# Autodesk Inventor assembly: Ensamblaje Alison Martínez 1190119
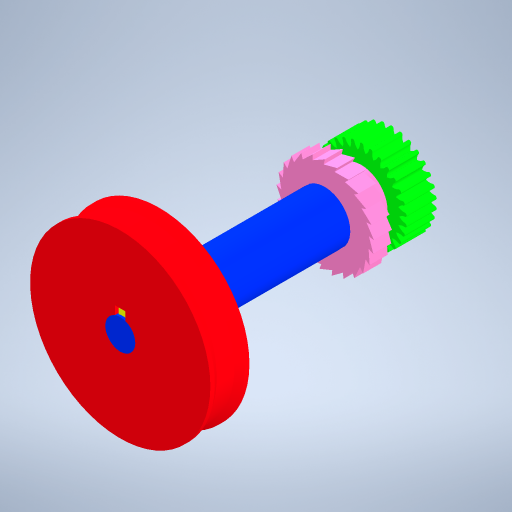
[picture p0: Inventor's stored thumbnail of the model, 512x512]
Saved by Autodesk Inventor 2024 (Build 280153000, 153)
## iProperties
Created: 2024-03-25
Part Number: Ensamblaje Alison Martínez 1190119
Document SubType Name: Assembly
Designer: Alison
Author: Alison
## Documents named in this file (6)
- C:\Users\Alison\Documents\Inventario\Ensamblaje Alison Martínez 1190119.iam
- C:\Users\Alison\Downloads\POLEA.ipt
- C:\Users\Alison\Downloads\ENGRANE.ipt
- C:\Users\Alison\Downloads\EJE_CUÑEROS.ipt
- C:\Users\Alison\Downloads\CUÑA.ipt
- C:\Users\Alison\Documents\Inventario\Pieza Creada - Alison.ipt
## Components (6 placed, 5 different names)
1. CUÑA:1 — Plana:2, Coincidencia:3, Coincidencia:4
2. EJE_CUÑEROS:1 — Cilíndrica:1, Cilíndrica:2, Nivelación:1, Cilíndrica:3, Nivelación:2, Plana:1, Coincidencia:1, Coincidencia:2, Plana:2, Coincidencia:3, Coincidencia:4, Rígido:5
3. ENGRANE:1 — Cilíndrica:3, Nivelación:2
4. POLEA:1 — Cilíndrica:1, Cilíndrica:2, Nivelación:1
5. CUÑA:2 — Plana:1, Coincidencia:1, Coincidencia:2
6. Pieza Creada - Alison:1 — Rígido:5
## Relationships (12: Mate 4, CylindricalJoint 3, Flush 2, PlanarJoint 2, WeldJoint 1)
- Cilíndrica:1 [CylindricalJoint]: EJE_CUÑEROS:1 ↔ POLEA:1
- Cilíndrica:2 [CylindricalJoint]: EJE_CUÑEROS:1 ↔ POLEA:1
- Nivelación:1 [Flush]: EJE_CUÑEROS:1 ↔ POLEA:1
- Cilíndrica:3 [CylindricalJoint]: EJE_CUÑEROS:1 ↔ ENGRANE:1
- Nivelación:2 [Flush] (8.6 mm): EJE_CUÑEROS:1 ↔ ENGRANE:1
- Plana:1: EJE_CUÑEROS:1 ↔ CUÑA:2
- Coincidencia:1 [Mate]: EJE_CUÑEROS:1 ↔ CUÑA:2
- Coincidencia:2 [Mate]: EJE_CUÑEROS:1 ↔ CUÑA:2
- Plana:2: CUÑA:1 ↔ EJE_CUÑEROS:1
- Coincidencia:3 [Mate]: CUÑA:1 ↔ EJE_CUÑEROS:1
- Coincidencia:4 [Mate]: CUÑA:1 ↔ EJE_CUÑEROS:1
- Rígido:5 [WeldJoint] (-2.8 mm): EJE_CUÑEROS:1 ↔ Pieza Creada - Alison:1
